# Autodesk Inventor assembly: Piston rod
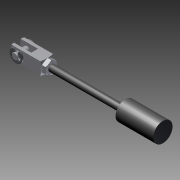
[picture p0: Inventor's stored thumbnail of the model, 180x180]
Saved by Autodesk Inventor 2012 (Build 160160000, 160)
## iProperties
Created: 2013-01-19
Part Number: Piston rod
Document SubType Name: Assembly
Designer: William
Mass: 17.4918 g
Surface Area: 79.8005 cm^2
Volume: 17.4918 cm^3
Density: 1 g/cm^3
Author: William
## Documents named in this file (6)
- Z:\UserData\Documents\Inventor\team1885frc\Robot2013\Launcher\Piston\2inch\Piston rod.iam
- Z:\UserData\Documents\Inventor\team1885frc\Robot2013\Launcher\Piston\2inch\0420_rod.ipt
- Z:\UserData\Documents\Inventor\team1885frc\Robot2013\Launcher\Piston\.75 inch\D-14055.ipt
- Z:\UserData\Documents\Inventor\team1885frc\Robot2013\Launcher\Piston\.75 inch\D-8381.ipt
- Z:\UserData\Documents\Inventor\team1885frc\Robot2013\Launcher\Piston\.75 inch\D-5866.ipt
- Z:\UserData\Documents\Inventor\team1885frc\Robot2013\Launcher\Piston\.75 inch\D-344.ipt
## Components (6 placed, 5 different names)
1. 0420_rod:1 — Mate:9, Flush:1
2. D-14055:1 — Mate:1, Mate:2, Mate:7, Mate:8
3. D-8381:1 — Mate:1, Mate:3, Mate:4, Mate:5, Mate:6
4. D-5866:1 — Mate:2, Mate:3, Mate:4
5. D-5866:2 — Mate:5, Mate:6
6. D-344:1 — Mate:7, Mate:8, Mate:9, Flush:1
## Relationships (10: Mate 9, Flush 1)
- Mate:1: D-14055:1 ↔ D-8381:1
- Mate:2: D-14055:1 ↔ D-5866:1
- Mate:3: D-8381:1 ↔ D-5866:1
- Mate:4: D-8381:1 ↔ D-5866:1
- Mate:5: D-8381:1 ↔ D-5866:2
- Mate:6: D-8381:1 ↔ D-5866:2
- Mate:7: D-14055:1 ↔ D-344:1
- Mate:8: D-14055:1 ↔ D-344:1
- Mate:9: 0420_rod:1 ↔ D-344:1
- Flush:1: 0420_rod:1 ↔ D-344:1
